# Autodesk Inventor assembly: Bumper Piston
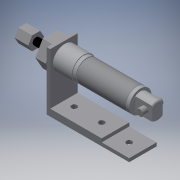
[picture p0: Inventor's stored thumbnail of the model, 180x180]
Saved by Autodesk Inventor 2018 (Build 220112000, 112)
## iProperties
Created: 2019-01-25
Part Number: Bumper Piston
Document SubType Name: Assembly
Designer: s-2512711
Author: s-2512711
## Documents named in this file (6)
- C:\Users\s-2512711\Desktop\Github\2019CAD\Drivebase but Calvin is a mad man\Bumper Piston.iam
- C:\Users\s-2512711\Desktop\Github\2019CAD\Drivebase but Calvin is a mad man\Piston bracket.ipt
- C:\Users\s-2512711\Desktop\Github\2019CAD\Drivebase but Calvin is a mad man\AIS2018\040_5-RP.iam
- C:\Users\s-2512711\Desktop\Github\2019CAD\Drivebase but Calvin is a mad man\Piston nut.ipt
- C:\Users\s-2512711\Desktop\Github\2019CAD\Drivebase but Calvin is a mad man\Piston Plate.ipt
- C:\Users\s-2512711\Desktop\Github\2019CAD\Drivebase but Calvin is a mad man\Piston Hex Shaft.ipt
## Components (5 placed, 5 different names)
1. Piston bracket:1 — Mate:1, Mate:2, Angle:1, Mate:3, Mate:5, Mate:6, Mate:7
2. 040_5-RP:1 [sub-assembly] — Mate:1, Mate:2, Angle:1, Mate:4, Mate:8, Flush:1
3. Piston nut:1 — Mate:3, Mate:4, Angle:2
4. Piston Plate:1 — Mate:5, Mate:6, Mate:7
5. Piston Hex Shaft:1 — Mate:8, Flush:1, Angle:2
## Relationships (11: Mate 8, Angle 2, Flush 1)
- Mate:1: Piston bracket:1 ↔ 040_5-RP:1
- Mate:2: Piston bracket:1 ↔ 040_5-RP:1
- Angle:1 (90 deg): Piston bracket:1 ↔ 040_5-RP:1
- Mate:3: Piston bracket:1 ↔ Piston nut:1
- Mate:4: 040_5-RP:1 ↔ Piston nut:1
- Mate:5: Piston bracket:1 ↔ Piston Plate:1
- Mate:6: Piston bracket:1 ↔ Piston Plate:1
- Mate:7: Piston bracket:1 ↔ Piston Plate:1
- Mate:8: 040_5-RP:1 ↔ Piston Hex Shaft:1
- Flush:1: 040_5-RP:1 ↔ Piston Hex Shaft:1
- Angle:2 (0 deg): Piston nut:1 ↔ Piston Hex Shaft:1
